# Autodesk Inventor assembly: Asem
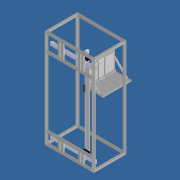
[picture p0: Inventor's stored thumbnail of the model, 180x180]
Saved by Autodesk Inventor 2020 (Build 240168000, 168)
## iProperties
Created: 2021-02-24
Part Number: Asem
Document SubType Name: Assembly
Designer: magnarecta
Author: magnarecta
## Documents named in this file (9)
- D:\Document\Github\Eto_Project\Hardware\Asem\Asem.iam
- D:\Document\Github\Eto_Project\Hardware\Parts\MISUMI\HFS6-3030-1500_Autodesk_Inventor_2020_20210225\HFS6-3030-1500.ipt
- D:\Document\Github\Eto_Project\Hardware\Parts\MISUMI\HFS6-3030-690_Autodesk_Inventor_2020_20210225\HFS6-3030-690.ipt
- D:\Document\Github\Eto_Project\Hardware\Parts\MISUMI\HFS6-3030-440_Autodesk_Inventor_2020_20210225\HFS6-3030-440.ipt
- D:\Document\Github\Eto_Project\Hardware\Asem\CCM_Unit.iam
- D:\Document\Github\Eto_Project\Hardware\Parts\MISUMI\HFS6-3030-223_Autodesk_Inventor_2020_20210225\HFS6-3030-223.ipt
- D:\Document\Github\Eto_Project\Hardware\Parts\MISUMI\HFS6-3030-140_Autodesk_Inventor_2020_20210225\HFS6-3030-140.ipt
- D:\Document\Github\Eto_Project\Hardware\Parts\Meviy\Dragchain_Guide.ipt
- D:\Document\Github\Eto_Project\Hardware\Asem\Display_Unit.iam
## Components (26 placed, 8 different names)
1. HFS6-3030-1500:1 — フラッシュ:1, フラッシュ:2, フラッシュ:5, メイト:1, フラッシュ:6, フラッシュ:7, メイト:2, フラッシュ:9, フラッシュ:10, フラッシュ:18, フラッシュ:21, フラッシュ:25, メイト:20
2. HFS6-3030-1500:2 — フラッシュ:2, フラッシュ:5, メイト:1, フラッシュ:8, メイト:3, メイト:4, フラッシュ:11, フラッシュ:12, フラッシュ:20, メイト:10, フラッシュ:24, メイト:12, メイト:13, フラッシュ:26
3. HFS6-3030-1500:3 — フラッシュ:3, フラッシュ:4, フラッシュ:8, メイト:5, フラッシュ:13, フラッシュ:14, メイト:6, フラッシュ:15, フラッシュ:16
4. HFS6-3030-1500:4 — フラッシュ:1, フラッシュ:3, フラッシュ:4, フラッシュ:6, フラッシュ:7, メイト:2
5. HFS6-3030-690:1 — メイト:3, フラッシュ:9, フラッシュ:10, メイト:7, フラッシュ:17, メイト:8, フラッシュ:19, メイト:15, メイト:18, フラッシュ:33, メイト:19
6. HFS6-3030-690:2 — メイト:4, フラッシュ:11, フラッシュ:12, メイト:9, フラッシュ:22, フラッシュ:23, メイト:11, 角度:1, メイト:14, フラッシュ:28
7. HFS6-3030-690:3 — メイト:5, フラッシュ:13, フラッシュ:14
8. HFS6-3030-690:4 — メイト:6, フラッシュ:15, フラッシュ:16
9. HFS6-3030-440:1 — メイト:7, フラッシュ:17, フラッシュ:20
10. HFS6-3030-440:2 — メイト:8, フラッシュ:18, フラッシュ:19
11. HFS6-3030-440:3 — メイト:9, フラッシュ:21, フラッシュ:22
12. HFS6-3030-440:4 — メイト:10, フラッシュ:23, フラッシュ:24
13. CCM_Unit:1 [sub-assembly] — メイト:11, 角度:1, フラッシュ:27, フラッシュ:34, フラッシュ:36, メイト:24, メイト:25, メイト:26
14. HFS6-3030-690:5 — メイト:12, フラッシュ:25, メイト:14, フラッシュ:43, メイト:21
15. HFS6-3030-690:6 — メイト:13, フラッシュ:26, メイト:15, フラッシュ:35
16. HFS6-3030-223:1 — フラッシュ:31, フラッシュ:32, メイト:17, メイト:18, フラッシュ:47
17. HFS6-3030-223:2 — フラッシュ:31, フラッシュ:32, メイト:17, フラッシュ:33, フラッシュ:34, メイト:20, フラッシュ:44
18. HFS6-3030-223:3 — フラッシュ:29, フラッシュ:30, メイト:16, フラッシュ:46
19. HFS6-3030-223:4 — フラッシュ:29, フラッシュ:30, メイト:16, メイト:19, フラッシュ:35, フラッシュ:36, フラッシュ:45
20. HFS6-3030-140:1 — フラッシュ:37, フラッシュ:42, メイト:21, フラッシュ:44
21. HFS6-3030-140:2 — フラッシュ:37, フラッシュ:38, フラッシュ:41, フラッシュ:42, フラッシュ:43, フラッシュ:46
22. HFS6-3030-140:3 — フラッシュ:38, フラッシュ:39, フラッシュ:40, フラッシュ:41, フラッシュ:47
23. HFS6-3030-140:4 — フラッシュ:39, フラッシュ:40, フラッシュ:45
24. Dragchain_Guide:1 — メイト:23, フラッシュ:50, メイト:24, フラッシュ:51
25. Dragchain_Guide:3 — メイト:23, フラッシュ:50, フラッシュ:51, メイト:25, メイト:26
26. Display_Unit:1 [sub-assembly]
## Relationships (75: Flush 49, Mate 25, Angle 1)
- フラッシュ:1 [Flush]: HFS6-3030-1500:1 ↔ HFS6-3030-1500:4
- フラッシュ:2 [Flush]: HFS6-3030-1500:1 ↔ HFS6-3030-1500:2
- フラッシュ:3 [Flush]: HFS6-3030-1500:3 ↔ HFS6-3030-1500:4
- フラッシュ:4 [Flush]: HFS6-3030-1500:3 ↔ HFS6-3030-1500:4
- フラッシュ:5 [Flush]: HFS6-3030-1500:1 ↔ HFS6-3030-1500:2
- メイト:1 [Mate] (-750 mm): HFS6-3030-1500:1 ↔ HFS6-3030-1500:2
- フラッシュ:6 [Flush]: HFS6-3030-1500:1 ↔ HFS6-3030-1500:4
- フラッシュ:7 [Flush]: HFS6-3030-1500:1 ↔ HFS6-3030-1500:4
- フラッシュ:8 [Flush]: HFS6-3030-1500:2 ↔ HFS6-3030-1500:3
- メイト:2 [Mate] (-500 mm): HFS6-3030-1500:1 ↔ HFS6-3030-1500:4
- メイト:3 [Mate]: HFS6-3030-1500:2 ↔ HFS6-3030-690:1
- フラッシュ:9 [Flush]: HFS6-3030-1500:1 ↔ HFS6-3030-690:1
- フラッシュ:10 [Flush]: HFS6-3030-1500:1 ↔ HFS6-3030-690:1
- メイト:4 [Mate]: HFS6-3030-1500:2 ↔ HFS6-3030-690:2
- フラッシュ:11 [Flush]: HFS6-3030-1500:2 ↔ HFS6-3030-690:2
- フラッシュ:12 [Flush]: HFS6-3030-1500:2 ↔ HFS6-3030-690:2
- メイト:5 [Mate]: HFS6-3030-1500:3 ↔ HFS6-3030-690:3
- フラッシュ:13 [Flush]: HFS6-3030-1500:3 ↔ HFS6-3030-690:3
- フラッシュ:14 [Flush]: HFS6-3030-1500:3 ↔ HFS6-3030-690:3
- メイト:6 [Mate]: HFS6-3030-1500:3 ↔ HFS6-3030-690:4
- フラッシュ:15 [Flush]: HFS6-3030-1500:3 ↔ HFS6-3030-690:4
- フラッシュ:16 [Flush]: HFS6-3030-1500:3 ↔ HFS6-3030-690:4
- メイト:7 [Mate]: HFS6-3030-690:1 ↔ HFS6-3030-440:1
- フラッシュ:17 [Flush]: HFS6-3030-690:1 ↔ HFS6-3030-440:1
- メイト:8 [Mate]: HFS6-3030-690:1 ↔ HFS6-3030-440:2
- フラッシュ:18 [Flush]: HFS6-3030-1500:1 ↔ HFS6-3030-440:2
- フラッシュ:19 [Flush]: HFS6-3030-690:1 ↔ HFS6-3030-440:2
- フラッシュ:20 [Flush]: HFS6-3030-1500:2 ↔ HFS6-3030-440:1
- メイト:9 [Mate]: HFS6-3030-690:2 ↔ HFS6-3030-440:3
- フラッシュ:21 [Flush]: HFS6-3030-1500:1 ↔ HFS6-3030-440:3
- フラッシュ:22 [Flush]: HFS6-3030-690:2 ↔ HFS6-3030-440:3
- メイト:10 [Mate]: HFS6-3030-1500:2 ↔ HFS6-3030-440:4
- フラッシュ:23 [Flush]: HFS6-3030-690:2 ↔ HFS6-3030-440:4
- フラッシュ:24 [Flush]: HFS6-3030-1500:2 ↔ HFS6-3030-440:4
- メイト:11 [Mate] (2 mm): HFS6-3030-690:2 ↔ CCM_Unit:1
- 角度:1 [Angle] (0 deg): HFS6-3030-690:2 ↔ CCM_Unit:1
- メイト:12 [Mate]: HFS6-3030-1500:2 ↔ HFS6-3030-690:5
- フラッシュ:25 [Flush]: HFS6-3030-1500:1 ↔ HFS6-3030-690:5
- メイト:13 [Mate]: HFS6-3030-1500:2 ↔ HFS6-3030-690:6
- フラッシュ:26 [Flush]: HFS6-3030-1500:2 ↔ HFS6-3030-690:6
- メイト:14 [Mate] (-200 mm): HFS6-3030-690:2 ↔ HFS6-3030-690:5
- メイト:15 [Mate] (-283 mm): HFS6-3030-690:1 ↔ HFS6-3030-690:6
- フラッシュ:27 [Flush] (-10 mm): CCM_Unit:1
- フラッシュ:28 [Flush] (70 mm): HFS6-3030-690:2
- フラッシュ:29 [Flush]: HFS6-3030-223:3 ↔ HFS6-3030-223:4
- フラッシュ:30 [Flush]: HFS6-3030-223:3 ↔ HFS6-3030-223:4
- メイト:16 [Mate] (20 mm): HFS6-3030-223:3 ↔ HFS6-3030-223:4
- フラッシュ:31 [Flush]: HFS6-3030-223:1 ↔ HFS6-3030-223:2
- フラッシュ:32 [Flush]: HFS6-3030-223:1 ↔ HFS6-3030-223:2
- メイト:17 [Mate] (20 mm): HFS6-3030-223:1 ↔ HFS6-3030-223:2
- メイト:18 [Mate]: HFS6-3030-690:1 ↔ HFS6-3030-223:1
- フラッシュ:33 [Flush]: HFS6-3030-690:1 ↔ HFS6-3030-223:2
- フラッシュ:34 [Flush] (-7.5 mm): CCM_Unit:1 ↔ HFS6-3030-223:2
- メイト:19 [Mate]: HFS6-3030-690:1 ↔ HFS6-3030-223:4
- フラッシュ:35 [Flush]: HFS6-3030-690:6 ↔ HFS6-3030-223:4
- フラッシュ:36 [Flush]: CCM_Unit:1 ↔ HFS6-3030-223:4
- メイト:20 [Mate] (170 mm): HFS6-3030-1500:1 ↔ HFS6-3030-223:2
- フラッシュ:37 [Flush]: HFS6-3030-140:1 ↔ HFS6-3030-140:2
- フラッシュ:38 [Flush]: HFS6-3030-140:2 ↔ HFS6-3030-140:3
- フラッシュ:39 [Flush]: HFS6-3030-140:3 ↔ HFS6-3030-140:4
- フラッシュ:40 [Flush]: HFS6-3030-140:3 ↔ HFS6-3030-140:4
- フラッシュ:41 [Flush]: HFS6-3030-140:2 ↔ HFS6-3030-140:3
- フラッシュ:42 [Flush]: HFS6-3030-140:1 ↔ HFS6-3030-140:2
- フラッシュ:43 [Flush]: HFS6-3030-690:5 ↔ HFS6-3030-140:2
- メイト:21 [Mate]: HFS6-3030-690:5 ↔ HFS6-3030-140:1
- フラッシュ:44 [Flush]: HFS6-3030-223:2 ↔ HFS6-3030-140:1
- フラッシュ:45 [Flush]: HFS6-3030-223:4 ↔ HFS6-3030-140:4
- フラッシュ:46 [Flush]: HFS6-3030-223:3 ↔ HFS6-3030-140:2
- フラッシュ:47 [Flush]: HFS6-3030-223:1 ↔ HFS6-3030-140:3
- メイト:23 [Mate]: Dragchain_Guide:1 ↔ Dragchain_Guide:3
- フラッシュ:50 [Flush]: Dragchain_Guide:1 ↔ Dragchain_Guide:3
- メイト:24 [Mate]: CCM_Unit:1 ↔ Dragchain_Guide:1
- フラッシュ:51 [Flush]: Dragchain_Guide:1 ↔ Dragchain_Guide:3
- メイト:25 [Mate]: CCM_Unit:1 ↔ Dragchain_Guide:3
- メイト:26 [Mate] (-13 mm): CCM_Unit:1 ↔ Dragchain_Guide:3
